# Autodesk Inventor assembly: FrameV4
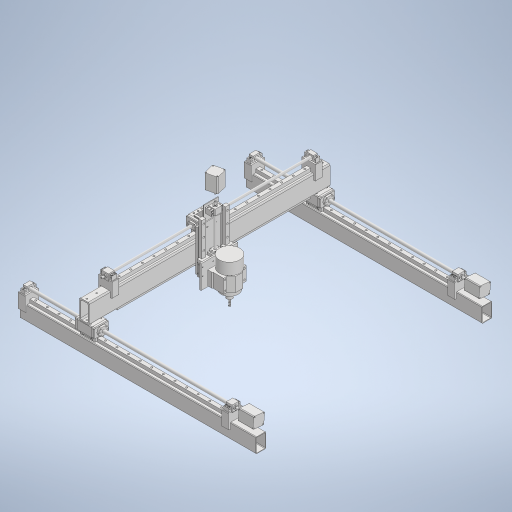
[picture p0: Inventor's stored thumbnail of the model, 512x512]
Saved by Autodesk Inventor 2023 (Build 270158000, 158)
## iProperties
Created: 2022-05-07
Part Number: FrameV4
Document SubType Name: Assembly
Designer: plebbb
Mass: 10930.1 g
Surface Area: 33660.3 cm^2
Volume: 10930.1 cm^3
Density: 1 g/cm^3
Author: plebbb
## Documents named in this file (24)
- D:\Users\plebbb\Desktop\CNC_Project\FrameV4.iam
- D:\Users\plebbb\Desktop\CNC_Project\X_GANTRY.iam
- D:\Users\plebbb\Desktop\CNC_Project\Ballscrew_Assembly.iam
- D:\Users\plebbb\Desktop\CNC_Project\2x4_Tube.ipt
- D:\Users\plebbb\Desktop\CNC_Project\HGW20CC_Rail_800mm.ipt
- D:\Users\plebbb\Desktop\CNC_Project\BK10.ipt
- D:\Users\plebbb\Desktop\CNC_Project\BF10.ipt
- D:\Users\plebbb\Desktop\CNC_Project\Ballscrew_Assembly_1204.iam
- D:\Users\plebbb\Desktop\CNC_Project\SFU1204-500.ipt
- D:\Users\plebbb\Desktop\CNC_Project\BF10_Spacer.ipt
- D:\Users\plebbb\Desktop\CNC_Project\BK10_Spacer.ipt
- D:\Users\plebbb\Desktop\CNC_Project\2x3_L_Bracket.ipt
- D:\Users\plebbb\Desktop\CNC_Project\HGW20CC_Slider.ipt
- D:\Users\plebbb\Desktop\CNC_Project\Z_Gantry_Plate.ipt
- D:\Users\plebbb\Desktop\CNC_Project\HGW20CC_Rail_300mm.ipt
- D:\Users\plebbb\Desktop\CNC_Project\Rail_Spacer_Plate.ipt
- D:\Users\plebbb\Desktop\CNC_Project\Z_PLATE.iam
- D:\Users\plebbb\Desktop\CNC_Project\SFU1204-300.ipt
- D:\Users\plebbb\Desktop\CNC_Project\Spindle.ipt
- D:\Users\plebbb\Desktop\CNC_Project\Spindle_Holder.ipt
- D:\Users\plebbb\Desktop\CNC_Project\BK10_Z_Mount.ipt
- D:\Users\plebbb\Desktop\CNC_Project\Corner_Brace.ipt
- D:\Users\plebbb\Desktop\CNC_Project\Nema23.ipt
- D:\Users\plebbb\Desktop\CNC_Project\Drill_Bit.ipt
## Components (30 placed, 23 different names)
1. X_GANTRY:1 [sub-assembly] — Mate:1, Mate:2, Flush:1, Flush:2, Flush:3, Mate:3, Mate:4, Mate:13, Mate:14
2. X_GANTRY:2 [sub-assembly] — Flush:2, Flush:3, Mate:5, Mate:6
3. Ballscrew_Assembly:1 [sub-assembly] — Mate:3, Mate:4, Mate:7, Mate:8, Mate:11, Mate:13, Mate:14
4. Ballscrew_Assembly:2 [sub-assembly] — Mate:5, Mate:6, Mate:9, Mate:10, Mate:12
5. 2x4_Tube:1 — Mate:7, Mate:8, Mate:9, Mate:10, Mate:11, Mate:12, Flush:4, Mate:15, Mate:26, Mate:27, Mate:34, Mate:35, Flush:5, Mate:45
6. HGW20CC_Rail_800mm:1 — Flush:4, Mate:15, Mate:22, Mate:23, Mate:38, Flush:6, Flush:7
7. BK10:1 — Mate:40, Mate:41, Mate:42, Mate:43, Mate:44
8. BF10:1 — Mate:31, Mate:32, Mate:33, Mate:36
9. Ballscrew_Assembly_1204:1 [sub-assembly] — Mate:22, Mate:23, Mate:24, Mate:39, Mate:44, Mate:51, Mate:52, Mate:54, Mate:68, Angle:3
10. SFU1204-500:1 — Mate:24, Mate:36, Mate:43
11. BF10_Spacer:1 — Mate:31, Mate:32, Mate:33, Mate:34, Mate:35, Flush:5, Mate:38, Mate:39
12. BK10_Spacer:1 — Mate:26, Mate:27, Mate:40, Mate:41, Mate:42
13. HGW20CC_Rail_800mm:2 — Flush:6, Mate:45, Mate:49, Mate:50, Flush:7
14. 2x3_L_Bracket:1 — Mate:46, Mate:47, Mate:48, Mate:53
15. HGW20CC_Slider:1 — Mate:46, Mate:47, Mate:48, Mate:49, Mate:50
16. Z_Gantry_Plate:1 — Mate:51, Mate:52, Mate:53, Mate:54, Angle:2, Mate:55, Mate:56, Flush:9, Flush:10, Flush:12, Flush:14, Flush:15, Flush:17
17. HGW20CC_Rail_300mm:1 — Flush:8, Angle:1, Angle:2, Mate:57, Flush:11, Flush:12, Flush:16
18. HGW20CC_Rail_300mm:2 — Flush:8, Angle:1, Mate:58, Flush:13, Flush:14, Flush:15, Mate:59, Mate:60
19. Rail_Spacer_Plate:1 — Mate:55, Flush:9, Mate:57, Flush:11
20. Rail_Spacer_Plate:2 — Mate:56, Flush:10, Mate:58, Flush:13
21. Z_PLATE:1 [sub-assembly] — Mate:59, Mate:60, Flush:16, Mate:61, Mate:63, Mate:64, Mate:65
22. SFU1204-300:1 — Mate:61, Flush:17, Mate:66, Mate:67, Mate:74
23. Spindle:1 — Mate:62, Flush:18, Mate:75, Mate:76
24. Spindle_Holder:1 — Mate:62, Flush:18, Mate:63, Mate:64, Mate:65
25. BK10:2 — Mate:66, Mate:67, Mate:69
26. BK10_Z_Mount:1 — Mate:68, Mate:69, Angle:3, Mate:70, Mate:71, Mate:72, Mate:73, Flush:19, Flush:20
27. Corner_Brace:1 — Mate:71, Mate:72, Flush:19
28. Corner_Brace:2 — Mate:70, Mate:73, Flush:20
29. Nema23:1 — Mate:74
30. Drill_Bit:1 — Mate:75, Mate:76
## Relationships (88: Mate 65, Flush 20, Angle 3)
- Mate:1: X_GANTRY:1
- Mate:2: X_GANTRY:1
- Flush:1: X_GANTRY:1
- Flush:2: X_GANTRY:1 ↔ X_GANTRY:2
- Flush:3: X_GANTRY:1 ↔ X_GANTRY:2
- Mate:3: X_GANTRY:1 ↔ Ballscrew_Assembly:1
- Mate:4: X_GANTRY:1 ↔ Ballscrew_Assembly:1
- Mate:5: X_GANTRY:2 ↔ Ballscrew_Assembly:2
- Mate:6: X_GANTRY:2 ↔ Ballscrew_Assembly:2
- Mate:7: Ballscrew_Assembly:1 ↔ 2x4_Tube:1
- Mate:8: Ballscrew_Assembly:1 ↔ 2x4_Tube:1
- Mate:9: Ballscrew_Assembly:2 ↔ 2x4_Tube:1
- Mate:10: Ballscrew_Assembly:2 ↔ 2x4_Tube:1
- Mate:11: Ballscrew_Assembly:1 ↔ 2x4_Tube:1
- Mate:12: Ballscrew_Assembly:2 ↔ 2x4_Tube:1
- Mate:13: X_GANTRY:1 ↔ Ballscrew_Assembly:1
- Mate:14: X_GANTRY:1 ↔ Ballscrew_Assembly:1
- Flush:4 (15.4 mm): 2x4_Tube:1 ↔ HGW20CC_Rail_800mm:1
- Mate:15: 2x4_Tube:1 ↔ HGW20CC_Rail_800mm:1
- Mate:22: HGW20CC_Rail_800mm:1 ↔ Ballscrew_Assembly_1204:1
- Mate:23: HGW20CC_Rail_800mm:1 ↔ Ballscrew_Assembly_1204:1
- Mate:24: Ballscrew_Assembly_1204:1 ↔ SFU1204-500:1
- Mate:26: 2x4_Tube:1 ↔ BK10_Spacer:1
- Mate:27: 2x4_Tube:1 ↔ BK10_Spacer:1
- Mate:31: BF10:1 ↔ BF10_Spacer:1
- Mate:32: BF10:1 ↔ BF10_Spacer:1
- Mate:33: BF10:1 ↔ BF10_Spacer:1
- Mate:34: 2x4_Tube:1 ↔ BF10_Spacer:1
- Mate:35: 2x4_Tube:1 ↔ BF10_Spacer:1
- Mate:36: BF10:1 ↔ SFU1204-500:1
- Flush:5 (50 mm): 2x4_Tube:1 ↔ BF10_Spacer:1
- Mate:38: HGW20CC_Rail_800mm:1 ↔ BF10_Spacer:1
- Mate:39: Ballscrew_Assembly_1204:1 ↔ BF10_Spacer:1
- Mate:40: BK10:1 ↔ BK10_Spacer:1
- Mate:41: BK10:1 ↔ BK10_Spacer:1
- Mate:42: BK10:1 ↔ BK10_Spacer:1
- Mate:43: BK10:1 ↔ SFU1204-500:1
- Mate:44: BK10:1 ↔ Ballscrew_Assembly_1204:1
- Flush:6: HGW20CC_Rail_800mm:1 ↔ HGW20CC_Rail_800mm:2
- Mate:45: 2x4_Tube:1 ↔ HGW20CC_Rail_800mm:2
- Mate:46: 2x3_L_Bracket:1 ↔ HGW20CC_Slider:1
- Mate:47: 2x3_L_Bracket:1 ↔ HGW20CC_Slider:1
- Mate:48: 2x3_L_Bracket:1 ↔ HGW20CC_Slider:1
- Mate:49: HGW20CC_Rail_800mm:2 ↔ HGW20CC_Slider:1
- Mate:50: HGW20CC_Rail_800mm:2 ↔ HGW20CC_Slider:1
- Flush:7: HGW20CC_Rail_800mm:1 ↔ HGW20CC_Rail_800mm:2
- Mate:51: Ballscrew_Assembly_1204:1 ↔ Z_Gantry_Plate:1
- Mate:52: Ballscrew_Assembly_1204:1 ↔ Z_Gantry_Plate:1
- Mate:53: 2x3_L_Bracket:1 ↔ Z_Gantry_Plate:1
- Mate:54: Ballscrew_Assembly_1204:1 ↔ Z_Gantry_Plate:1
- Flush:8: HGW20CC_Rail_300mm:1 ↔ HGW20CC_Rail_300mm:2
- Angle:1 (0 deg): HGW20CC_Rail_300mm:1 ↔ HGW20CC_Rail_300mm:2
- Angle:2 (0 deg): Z_Gantry_Plate:1 ↔ HGW20CC_Rail_300mm:1
- Mate:55: Z_Gantry_Plate:1 ↔ Rail_Spacer_Plate:1
- Mate:56: Z_Gantry_Plate:1 ↔ Rail_Spacer_Plate:2
- Flush:9: Z_Gantry_Plate:1 ↔ Rail_Spacer_Plate:1
- Flush:10: Z_Gantry_Plate:1 ↔ Rail_Spacer_Plate:2
- Mate:57: HGW20CC_Rail_300mm:1 ↔ Rail_Spacer_Plate:1
- Mate:58: HGW20CC_Rail_300mm:2 ↔ Rail_Spacer_Plate:2
- Flush:11: HGW20CC_Rail_300mm:1 ↔ Rail_Spacer_Plate:1
- Flush:12 (5.2 mm): Z_Gantry_Plate:1 ↔ HGW20CC_Rail_300mm:1
- Flush:13: HGW20CC_Rail_300mm:2 ↔ Rail_Spacer_Plate:2
- Flush:14 (5.2 mm): Z_Gantry_Plate:1 ↔ HGW20CC_Rail_300mm:2
- Flush:15: Z_Gantry_Plate:1 ↔ HGW20CC_Rail_300mm:2
- Mate:59: HGW20CC_Rail_300mm:2 ↔ Z_PLATE:1
- Mate:60: HGW20CC_Rail_300mm:2 ↔ Z_PLATE:1
- Flush:16: HGW20CC_Rail_300mm:1 ↔ Z_PLATE:1
- Mate:61: Z_PLATE:1 ↔ SFU1204-300:1
- Flush:17: Z_Gantry_Plate:1 ↔ SFU1204-300:1
- Mate:62: Spindle:1 ↔ Spindle_Holder:1
- Flush:18 (-20 mm): Spindle:1 ↔ Spindle_Holder:1
- Mate:63: Z_PLATE:1 ↔ Spindle_Holder:1
- Mate:64: Z_PLATE:1 ↔ Spindle_Holder:1
- Mate:65: Z_PLATE:1 ↔ Spindle_Holder:1
- Mate:66: SFU1204-300:1 ↔ BK10:2
- Mate:67: SFU1204-300:1 ↔ BK10:2
- Mate:68: Ballscrew_Assembly_1204:1 ↔ BK10_Z_Mount:1
- Mate:69: BK10:2 ↔ BK10_Z_Mount:1
- Angle:3 (180 deg): Ballscrew_Assembly_1204:1 ↔ BK10_Z_Mount:1
- Mate:70: BK10_Z_Mount:1 ↔ Corner_Brace:2
- Mate:71: BK10_Z_Mount:1 ↔ Corner_Brace:1
- Mate:72: BK10_Z_Mount:1 ↔ Corner_Brace:1
- Mate:73: BK10_Z_Mount:1 ↔ Corner_Brace:2
- Flush:19: BK10_Z_Mount:1 ↔ Corner_Brace:1
- Flush:20: BK10_Z_Mount:1 ↔ Corner_Brace:2
- Mate:74: SFU1204-300:1 ↔ Nema23:1
- Mate:75: Spindle:1 ↔ Drill_Bit:1
- Mate:76: Spindle:1 ↔ Drill_Bit:1
